# Autodesk Inventor assembly: ring-holder-one-sixth
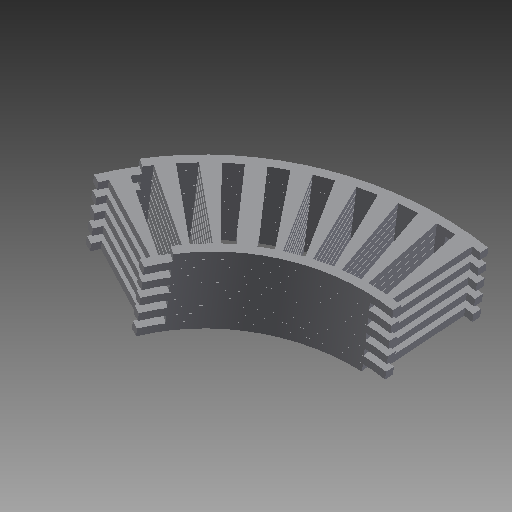
[picture p0: Inventor's stored thumbnail of the model, 512x512]
Saved by Autodesk Inventor 2018 (Build 220112000, 112)
## iProperties
Created: 2024-05-02
Part Number: ring-holder-one-sixth
Document SubType Name: Assembly
Designer: neo
Mass: 208.261 g
Surface Area: 1465 cm^2
Volume: 208.261 cm^3
Density: 1 g/cm^3
Author: neo
## Documents named in this file (2)
- D:\projects\kreion\design1\3d\ring-holder-one-sixth.iam
- D:\projects\kreion\design1\3d\ring-holder-one-sixth-2.iam
## Components (5 placed, 1 different names)
1. ring-holder-one-sixth-2:1 [sub-assembly] — Tangent:1, Tangent:2, Mate:1, Flush:1, Flush:2, Mate:2
2. ring-holder-one-sixth-2:2 [sub-assembly] — Tangent:1, Mate:1, Flush:1
3. ring-holder-one-sixth-2:3 [sub-assembly] — Tangent:2, Flush:2, Mate:2, Tangent:3, Flush:3, Mate:3, Tangent:4
4. ring-holder-one-sixth-2:4 [sub-assembly] — Tangent:3, Flush:3, Mate:3, Flush:4, Mate:4
5. ring-holder-one-sixth-2:5 [sub-assembly] — Tangent:4, Flush:4, Mate:4
## Relationships (12: Tangent 4, Mate 4, Flush 4)
- Tangent:1: ring-holder-one-sixth-2:1 ↔ ring-holder-one-sixth-2:2
- Tangent:2: ring-holder-one-sixth-2:1 ↔ ring-holder-one-sixth-2:3
- Mate:1: ring-holder-one-sixth-2:1 ↔ ring-holder-one-sixth-2:2
- Flush:1: ring-holder-one-sixth-2:1 ↔ ring-holder-one-sixth-2:2
- Flush:2: ring-holder-one-sixth-2:1 ↔ ring-holder-one-sixth-2:3
- Mate:2: ring-holder-one-sixth-2:1 ↔ ring-holder-one-sixth-2:3
- Tangent:3: ring-holder-one-sixth-2:3 ↔ ring-holder-one-sixth-2:4
- Flush:3: ring-holder-one-sixth-2:3 ↔ ring-holder-one-sixth-2:4
- Mate:3: ring-holder-one-sixth-2:3 ↔ ring-holder-one-sixth-2:4
- Tangent:4: ring-holder-one-sixth-2:3 ↔ ring-holder-one-sixth-2:5
- Flush:4: ring-holder-one-sixth-2:4 ↔ ring-holder-one-sixth-2:5
- Mate:4: ring-holder-one-sixth-2:4 ↔ ring-holder-one-sixth-2:5
